# Autodesk Inventor assembly: HexTrayRed
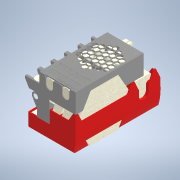
[picture p0: Inventor's stored thumbnail of the model, 180x180]
Saved by Autodesk Inventor 2021 (Build 250183000, 183)
## iProperties
Created: 2023-03-18
Part Number: HexTrayRed
Document SubType Name: Assembly
Designer: Bradley
Author: Bradley
## Documents named in this file (17)
- C:\Users\Bradley\Git\TI4\Hexes\HexTrayRed.iam
- C:\Users\Bradley\Git\TI4\Components\Hex_Hyperlanes_All.ipt
- C:\Users\Bradley\Git\TI4\Components\Hex_Mecatol.ipt
- C:\Users\Bradley\Git\TI4\Components\Hex_Reds_All.ipt
- C:\Users\Bradley\Git\TI4\Hexes\HexTrayRed.ipt
- C:\Users\Bradley\Git\TI4\Components\ActionCards_All.ipt
- C:\Users\Bradley\Git\TI4\Components\Exploration_SingleType.ipt
- C:\Users\Bradley\Git\TI4\Components\Objects_Public_SingleType.ipt
- C:\Users\Bradley\Git\TI4\Components\Objects_Secret_All.ipt
- C:\Users\Bradley\Git\TI4\Components\Relics_All.ipt
- C:\Users\Bradley\Git\TI4\Components\Planets_All.ipt
- C:\Users\Bradley\Git\TI4\Components\Agendas_All.ipt
- C:\Users\Bradley\Git\TI4\Hexes\HexTrayRed_Insert.ipt
- C:\Users\Bradley\Git\TI4\Hexes\CardboardTray.ipt
- C:\Users\Bradley\Git\TI4\Components\Cardboard_1_Single.ipt
- C:\Users\Bradley\Git\TI4\Components\Cardboard_3_Single.ipt
- C:\Users\Bradley\Git\TI4\Hexes\CardboardTray_Lid2.ipt
## Components (205 placed, 16 different names)
1. CardboardTray:1 — Mate:41, Flush:21, Flush:22, Insert:1, Insert:44, Insert:45, Insert:46, Insert:47, Insert:48, Insert:49, Mate:42, Mate:43, Mate:44, Mate:45, Mate:46, Mate:47, Mate:48, Mate:49, Mate:50, Mate:51, Mate:52, Mate:53, Mate:54, Mate:55, Mate:56, Mate:57, Mate:58, Mate:59, Mate:60, Mate:61, Mate:62
2. HexTrayRed:1 — Mate:2, Mate:3, Flush:3, Mate:4, Mate:11, Mate:12, Mate:13, Mate:16, Mate:17, Mate:18, Mate:19, Mate:20, Mate:21, Mate:22, Mate:23, Mate:24, Mate:25, Mate:26, Mate:27, Mate:28, Mate:29, Mate:30, Mate:31, Mate:32, Mate:33, Flush:20, Mate:34, Mate:41, Flush:21, Flush:22
3. HexTrayRed_Insert:1 — Mate:33, Flush:20, Mate:34, Mate:35, Mate:36, Mate:37, Mate:38, Mate:39, Mate:40
4. CardboardTray_Lid2:1 — Mate:60, Mate:61, Mate:62
5. Agendas_All:1 — Mate:36, Mate:37, Mate:39
6. ActionCards_All:1 — Mate:19, Mate:20, Mate:21
7. Hex_Hyperlanes_All:1 — Mate:1, Flush:1, Flush:2, Flush:4, Flush:5, Mate:4
8. Hex_Mecatol:1 — Mate:1, Flush:1, Flush:2
9. Hex_Reds_All:1 — Mate:2, Mate:3, Flush:3, Flush:4, Flush:5
10. Objects_Public_SingleType:1 — Mate:16, Mate:17, Mate:18
11. Objects_Public_SingleType:2
12. Objects_Secret_All:1
13. Planets_All:1 — Mate:35, Mate:38, Mate:40
14. Relics_All:1 — Mate:31, Mate:32, Flush:19
15. Cardboard_1_Single:1 — Insert:50, Mate:42
16. Cardboard_1_Single:10
17. Cardboard_1_Single:100
18. Cardboard_1_Single:101
19. Cardboard_1_Single:102
20. Cardboard_1_Single:103
21. Cardboard_1_Single:104 — Mate:54
22. Cardboard_1_Single:105
23. Cardboard_1_Single:106
24. Cardboard_1_Single:107
25. Cardboard_1_Single:108 — Insert:150
26. Cardboard_1_Single:109 — Insert:150
27. Cardboard_1_Single:11
28. Cardboard_1_Single:110
29. Cardboard_1_Single:111
30. Cardboard_1_Single:112
31. Cardboard_1_Single:113
32. Cardboard_1_Single:114 — Mate:58
33. Cardboard_1_Single:115
34. Cardboard_1_Single:116
35. Cardboard_1_Single:117
36. Cardboard_1_Single:118
37. Cardboard_1_Single:119 — Mate:59
38. Cardboard_1_Single:120
39. Cardboard_1_Single:121
40. Cardboard_1_Single:122
41. Cardboard_1_Single:123
42. Cardboard_1_Single:124 — Mate:56
43. Cardboard_1_Single:125
44. Cardboard_1_Single:126
45. Cardboard_1_Single:127
46. Cardboard_1_Single:128
47. Cardboard_1_Single:129
48. Cardboard_1_Single:13 — Mate:44
49. Cardboard_1_Single:130
50. Cardboard_1_Single:131
51. Cardboard_1_Single:132
52. Cardboard_1_Single:133
53. Cardboard_1_Single:134 — Mate:57
54. Cardboard_1_Single:135
55. Cardboard_1_Single:136
56. Cardboard_1_Single:137
57. Cardboard_1_Single:138
58. Cardboard_1_Single:139
59. Cardboard_1_Single:14
60. Cardboard_1_Single:140
61. Cardboard_1_Single:141
62. Cardboard_1_Single:142
63. Cardboard_1_Single:143
64. Cardboard_1_Single:15
65. Cardboard_1_Single:16
66. Cardboard_1_Single:17
67. Cardboard_1_Single:19 — Mate:47
68. Cardboard_1_Single:2 — Insert:50, Insert:51
69. Cardboard_1_Single:20
70. Cardboard_1_Single:21
71. Cardboard_1_Single:22
72. Cardboard_1_Single:23
73. Cardboard_1_Single:25 — Mate:46
74. Cardboard_1_Single:26
75. Cardboard_1_Single:27
76. Cardboard_1_Single:28
77. Cardboard_1_Single:29
78. Cardboard_1_Single:3 — Insert:51, Insert:52
79. Cardboard_1_Single:31 — Mate:45
80. Cardboard_1_Single:32
81. Cardboard_1_Single:33
82. Cardboard_1_Single:34
83. Cardboard_1_Single:35
84. Cardboard_1_Single:37 — Mate:48
85. Cardboard_1_Single:38
86. Cardboard_1_Single:39
87. Cardboard_1_Single:4 — Insert:52, Insert:53
88. Cardboard_1_Single:40
89. Cardboard_1_Single:41
90. Cardboard_1_Single:43 — Mate:49
91. Cardboard_1_Single:44
92. Cardboard_1_Single:45
93. Cardboard_1_Single:46
94. Cardboard_1_Single:47
95. Cardboard_1_Single:49 — Mate:50
96. Cardboard_1_Single:5 — Insert:53
97. Cardboard_1_Single:50
98. Cardboard_1_Single:51
99. Cardboard_1_Single:52
100. Cardboard_1_Single:53
101. Cardboard_1_Single:54 — Mate:51
102. Cardboard_1_Single:55
103. Cardboard_1_Single:56
104. Cardboard_1_Single:57
105. Cardboard_1_Single:58 — Insert:104
106. Cardboard_1_Single:59 — Insert:105, Insert:106
107. Cardboard_1_Single:60 — Insert:104
108. Cardboard_1_Single:61
109. Cardboard_1_Single:62
110. Cardboard_1_Single:63
111. Cardboard_1_Single:64 — Insert:105
112. Cardboard_1_Single:65 — Insert:106, Insert:107
113. Cardboard_1_Single:66 — Insert:107, Insert:108
114. Cardboard_1_Single:67 — Insert:108, Insert:109
115. Cardboard_1_Single:68 — Insert:109
116. Cardboard_1_Single:69 — Mate:53
117. Cardboard_1_Single:7 — Mate:43
118. Cardboard_1_Single:70
119. Cardboard_1_Single:71
120. Cardboard_1_Single:72
121. Cardboard_1_Single:73
122. Cardboard_1_Single:74
123. Cardboard_1_Single:75
124. Cardboard_1_Single:76
125. Cardboard_1_Single:77
126. Cardboard_1_Single:78
127. Cardboard_1_Single:79
128. Cardboard_1_Single:8
129. Cardboard_1_Single:80
130. Cardboard_1_Single:81
131. Cardboard_1_Single:82
132. Cardboard_1_Single:83
133. Cardboard_1_Single:84 — Mate:52
134. Cardboard_1_Single:85
135. Cardboard_1_Single:86
136. Cardboard_1_Single:87
137. Cardboard_1_Single:88
138. Cardboard_1_Single:89
139. Cardboard_1_Single:9
140. Cardboard_1_Single:90
141. Cardboard_1_Single:91
142. Cardboard_1_Single:92
143. Cardboard_1_Single:93
144. Cardboard_1_Single:94
145. Cardboard_1_Single:95
146. Cardboard_1_Single:96
147. Cardboard_1_Single:97
148. Cardboard_1_Single:98
149. Cardboard_1_Single:99 — Mate:55
150. Cardboard_3_Single:1 — Insert:1, Insert:2
151. Cardboard_3_Single:10
152. Cardboard_3_Single:11
153. Cardboard_3_Single:12
154. Cardboard_3_Single:13
155. Cardboard_3_Single:14
156. Cardboard_3_Single:15
157. Cardboard_3_Single:16
158. Cardboard_3_Single:17 — Insert:45
159. Cardboard_3_Single:18
160. Cardboard_3_Single:19
161. Cardboard_3_Single:2 — Insert:2, Insert:3
162. Cardboard_3_Single:20
163. Cardboard_3_Single:21
164. Cardboard_3_Single:22
165. Cardboard_3_Single:23
166. Cardboard_3_Single:24
167. Cardboard_3_Single:25 — Insert:46
168. Cardboard_3_Single:26
169. Cardboard_3_Single:27
170. Cardboard_3_Single:28
171. Cardboard_3_Single:29
172. Cardboard_3_Single:3 — Insert:3, Insert:4
173. Cardboard_3_Single:30
174. Cardboard_3_Single:31
175. Cardboard_3_Single:32
176. Cardboard_3_Single:33 — Insert:47
177. Cardboard_3_Single:34
178. Cardboard_3_Single:35
179. Cardboard_3_Single:36
180. Cardboard_3_Single:37
181. Cardboard_3_Single:38
182. Cardboard_3_Single:39
183. Cardboard_3_Single:4 — Insert:4, Insert:5
184. Cardboard_3_Single:40
185. Cardboard_3_Single:41 — Insert:55
186. Cardboard_3_Single:42 — Insert:55
187. Cardboard_3_Single:43
188. Cardboard_3_Single:44 — Insert:48
189. Cardboard_3_Single:46 — Insert:56
190. Cardboard_3_Single:47
191. Cardboard_3_Single:48 — Insert:49
192. Cardboard_3_Single:49 — Insert:56
193. Cardboard_3_Single:5 — Insert:5, Insert:6
194. Cardboard_3_Single:6 — Insert:6, Insert:7
195. Cardboard_3_Single:7 — Insert:7, Insert:8
196. Cardboard_3_Single:8 — Insert:8
197. Cardboard_3_Single:9 — Insert:44
198. Exploration_SingleType:1 — Mate:11, Mate:12, Mate:13
199. Exploration_SingleType:2
200. Exploration_SingleType:3
201. Exploration_SingleType:4
202. Exploration_SingleType:5 — Mate:22, Mate:23, Mate:24, Flush:16
203. Exploration_SingleType:6 — Mate:25, Mate:26, Flush:16, Flush:17
204. Exploration_SingleType:7 — Mate:27, Mate:28, Flush:17, Flush:18
205. Exploration_SingleType:8 — Mate:29, Mate:30, Flush:18, Flush:19
## Relationships (246: Insert 165, Mate 59, Flush 22)
- Mate:1: Hex_Hyperlanes_All:1 ↔ Hex_Mecatol:1
- Flush:1: Hex_Hyperlanes_All:1 ↔ Hex_Mecatol:1
- Flush:2: Hex_Hyperlanes_All:1 ↔ Hex_Mecatol:1
- Mate:2 (0.3 mm): HexTrayRed:1 ↔ Hex_Reds_All:1
- Mate:3: HexTrayRed:1 ↔ Hex_Reds_All:1
- Flush:3: HexTrayRed:1 ↔ Hex_Reds_All:1
- Flush:4: Hex_Hyperlanes_All:1 ↔ Hex_Reds_All:1
- Flush:5: Hex_Hyperlanes_All:1 ↔ Hex_Reds_All:1
- Mate:4 (0.4 mm): HexTrayRed:1 ↔ Hex_Hyperlanes_All:1
- [Mate]: Exploration_SingleType:1 ↔ Exploration_SingleType:2
- [Mate]: Exploration_SingleType:2 ↔ Exploration_SingleType:3
- [Mate]: Exploration_SingleType:3 ↔ Exploration_SingleType:4
- [Flush]: Exploration_SingleType:3 ↔ Exploration_SingleType:4
- [Flush]: Exploration_SingleType:2 ↔ Exploration_SingleType:3
- [Flush]: Exploration_SingleType:1 ↔ Exploration_SingleType:2
- [Flush]: Exploration_SingleType:3 ↔ Exploration_SingleType:4
- [Flush]: Exploration_SingleType:2 ↔ Exploration_SingleType:3
- [Flush]: Exploration_SingleType:1 ↔ Exploration_SingleType:2
- Mate:11: HexTrayRed:1 ↔ Exploration_SingleType:1
- Mate:12 (0.5 mm): HexTrayRed:1 ↔ Exploration_SingleType:1
- Mate:13 (0.5 mm): HexTrayRed:1 ↔ Exploration_SingleType:1
- [Mate]: Objects_Public_SingleType:1 ↔ Objects_Public_SingleType:2
- [Mate]: Objects_Public_SingleType:2 ↔ Objects_Secret_All:1
- [Flush]: Objects_Public_SingleType:2 ↔ Objects_Secret_All:1
- [Flush]: Objects_Public_SingleType:1 ↔ Objects_Public_SingleType:2
- [Flush]: Objects_Public_SingleType:1 ↔ Objects_Public_SingleType:2
- [Flush]: Objects_Public_SingleType:2 ↔ Objects_Secret_All:1
- Mate:16: HexTrayRed:1 ↔ Objects_Public_SingleType:1
- Mate:17 (0.5 mm): HexTrayRed:1 ↔ Objects_Public_SingleType:1
- Mate:18 (0.5 mm): HexTrayRed:1 ↔ Objects_Public_SingleType:1
- Mate:19: HexTrayRed:1 ↔ ActionCards_All:1
- Mate:20 (0.5 mm): HexTrayRed:1 ↔ ActionCards_All:1
- Mate:21 (0.5 mm): HexTrayRed:1 ↔ ActionCards_All:1
- Mate:22: HexTrayRed:1 ↔ Exploration_SingleType:5
- Mate:23: HexTrayRed:1 ↔ Exploration_SingleType:5
- Mate:24 (0.5 mm): HexTrayRed:1 ↔ Exploration_SingleType:5
- Mate:25: HexTrayRed:1 ↔ Exploration_SingleType:6
- Mate:26: HexTrayRed:1 ↔ Exploration_SingleType:6
- Mate:27: HexTrayRed:1 ↔ Exploration_SingleType:7
- Mate:28: HexTrayRed:1 ↔ Exploration_SingleType:7
- Mate:29: HexTrayRed:1 ↔ Exploration_SingleType:8
- Mate:30: HexTrayRed:1 ↔ Exploration_SingleType:8
- Flush:16: Exploration_SingleType:5 ↔ Exploration_SingleType:6
- Flush:17: Exploration_SingleType:6 ↔ Exploration_SingleType:7
- Flush:18: Exploration_SingleType:7 ↔ Exploration_SingleType:8
- Mate:31: HexTrayRed:1 ↔ Relics_All:1
- Mate:32: HexTrayRed:1 ↔ Relics_All:1
- Flush:19: Relics_All:1 ↔ Exploration_SingleType:8
- Mate:33: HexTrayRed:1 ↔ HexTrayRed_Insert:1
- Flush:20: HexTrayRed:1 ↔ HexTrayRed_Insert:1
- Mate:34: HexTrayRed:1 ↔ HexTrayRed_Insert:1
- Mate:35: HexTrayRed_Insert:1 ↔ Planets_All:1
- Mate:36: HexTrayRed_Insert:1 ↔ Agendas_All:1
- Mate:37: HexTrayRed_Insert:1 ↔ Agendas_All:1
- Mate:38: HexTrayRed_Insert:1 ↔ Planets_All:1
- Mate:39 (0.5 mm): HexTrayRed_Insert:1 ↔ Agendas_All:1
- Mate:40 (0.5 mm): HexTrayRed_Insert:1 ↔ Planets_All:1
- Mate:41: CardboardTray:1 ↔ HexTrayRed:1
- Flush:21: CardboardTray:1 ↔ HexTrayRed:1
- Flush:22: CardboardTray:1 ↔ HexTrayRed:1
- Insert:1: CardboardTray:1 ↔ Cardboard_3_Single:1
- Insert:2: Cardboard_3_Single:1 ↔ Cardboard_3_Single:2
- Insert:3: Cardboard_3_Single:2 ↔ Cardboard_3_Single:3
- Insert:4: Cardboard_3_Single:3 ↔ Cardboard_3_Single:4
- Insert:5: Cardboard_3_Single:4 ↔ Cardboard_3_Single:5
- Insert:6: Cardboard_3_Single:5 ↔ Cardboard_3_Single:6
- Insert:7: Cardboard_3_Single:6 ↔ Cardboard_3_Single:7
- Insert:8: Cardboard_3_Single:7 ↔ Cardboard_3_Single:8
- [Insert]: Cardboard_3_Single:10 ↔ Cardboard_3_Single:9
- [Insert]: Cardboard_3_Single:10 ↔ Cardboard_3_Single:11
- [Insert]: Cardboard_3_Single:11 ↔ Cardboard_3_Single:12
- [Insert]: Cardboard_3_Single:12 ↔ Cardboard_3_Single:13
- [Insert]: Cardboard_3_Single:13 ↔ Cardboard_3_Single:14
- [Insert]: Cardboard_3_Single:14 ↔ Cardboard_3_Single:15
- [Insert]: Cardboard_3_Single:15 ↔ Cardboard_3_Single:16
- [Insert]: Cardboard_3_Single:17 ↔ Cardboard_3_Single:18
- [Insert]: Cardboard_3_Single:18 ↔ Cardboard_3_Single:19
- [Insert]: Cardboard_3_Single:19 ↔ Cardboard_3_Single:20
- [Insert]: Cardboard_3_Single:20 ↔ Cardboard_3_Single:21
- [Insert]: Cardboard_3_Single:21 ↔ Cardboard_3_Single:22
- [Insert]: Cardboard_3_Single:22 ↔ Cardboard_3_Single:23
- [Insert]: Cardboard_3_Single:23 ↔ Cardboard_3_Single:24
- [Insert]: Cardboard_3_Single:25 ↔ Cardboard_3_Single:26
- [Insert]: Cardboard_3_Single:26 ↔ Cardboard_3_Single:27
- [Insert]: Cardboard_3_Single:27 ↔ Cardboard_3_Single:28
- [Insert]: Cardboard_3_Single:28 ↔ Cardboard_3_Single:29
- [Insert]: Cardboard_3_Single:29 ↔ Cardboard_3_Single:30
- [Insert]: Cardboard_3_Single:30 ↔ Cardboard_3_Single:31
- [Insert]: Cardboard_3_Single:31 ↔ Cardboard_3_Single:32
- [Insert]: Cardboard_3_Single:33 ↔ Cardboard_3_Single:34
- [Insert]: Cardboard_3_Single:34 ↔ Cardboard_3_Single:35
- [Insert]: Cardboard_3_Single:35 ↔ Cardboard_3_Single:36
- [Insert]: Cardboard_3_Single:36 ↔ Cardboard_3_Single:37
- [Insert]: Cardboard_3_Single:37 ↔ Cardboard_3_Single:38
- [Insert]: Cardboard_3_Single:38 ↔ Cardboard_3_Single:39
- [Insert]: Cardboard_3_Single:39 ↔ Cardboard_3_Single:40
- [Insert]: Cardboard_3_Single:42 ↔ Cardboard_3_Single:43
- [Insert]: Cardboard_3_Single:43 ↔ Cardboard_3_Single:44
- [Insert]: Cardboard_3_Single:46 ↔ Cardboard_3_Single:47
- [Insert]: Cardboard_3_Single:47 ↔ Cardboard_3_Single:48
- Insert:44: CardboardTray:1 ↔ Cardboard_3_Single:9
- Insert:45: CardboardTray:1 ↔ Cardboard_3_Single:17
- Insert:46: CardboardTray:1 ↔ Cardboard_3_Single:25
- Insert:47: CardboardTray:1 ↔ Cardboard_3_Single:33
- Insert:48 (0.5 mm): CardboardTray:1 ↔ Cardboard_3_Single:44
- Insert:49 (0.5 mm): CardboardTray:1 ↔ Cardboard_3_Single:48
- Insert:50: Cardboard_1_Single:1 ↔ Cardboard_1_Single:2
- Insert:51: Cardboard_1_Single:2 ↔ Cardboard_1_Single:3
- Insert:52: Cardboard_1_Single:3 ↔ Cardboard_1_Single:4
- Insert:53: Cardboard_1_Single:4 ↔ Cardboard_1_Single:5
- Insert:55: Cardboard_3_Single:41 ↔ Cardboard_3_Single:42
- Insert:56: Cardboard_3_Single:46 ↔ Cardboard_3_Single:49
- Mate:42: CardboardTray:1 ↔ Cardboard_1_Single:1
- [Insert]: Cardboard_1_Single:7 ↔ Cardboard_1_Single:8
- [Insert]: Cardboard_1_Single:8 ↔ Cardboard_1_Single:9
- [Insert]: Cardboard_1_Single:10 ↔ Cardboard_1_Single:9
- [Insert]: Cardboard_1_Single:10 ↔ Cardboard_1_Single:11
- [Insert]: Cardboard_1_Single:13 ↔ Cardboard_1_Single:14
- [Insert]: Cardboard_1_Single:14 ↔ Cardboard_1_Single:15
- [Insert]: Cardboard_1_Single:15 ↔ Cardboard_1_Single:16
- [Insert]: Cardboard_1_Single:16 ↔ Cardboard_1_Single:17
- [Insert]: Cardboard_1_Single:19 ↔ Cardboard_1_Single:20
- [Insert]: Cardboard_1_Single:20 ↔ Cardboard_1_Single:21
- [Insert]: Cardboard_1_Single:21 ↔ Cardboard_1_Single:22
- [Insert]: Cardboard_1_Single:22 ↔ Cardboard_1_Single:23
- [Insert]: Cardboard_1_Single:25 ↔ Cardboard_1_Single:26
- [Insert]: Cardboard_1_Single:26 ↔ Cardboard_1_Single:27
- [Insert]: Cardboard_1_Single:27 ↔ Cardboard_1_Single:28
- [Insert]: Cardboard_1_Single:28 ↔ Cardboard_1_Single:29
- [Insert]: Cardboard_1_Single:31 ↔ Cardboard_1_Single:32
- [Insert]: Cardboard_1_Single:32 ↔ Cardboard_1_Single:33
- [Insert]: Cardboard_1_Single:33 ↔ Cardboard_1_Single:34
- [Insert]: Cardboard_1_Single:34 ↔ Cardboard_1_Single:35
- [Insert]: Cardboard_1_Single:37 ↔ Cardboard_1_Single:38
- [Insert]: Cardboard_1_Single:38 ↔ Cardboard_1_Single:39
- [Insert]: Cardboard_1_Single:39 ↔ Cardboard_1_Single:40
- [Insert]: Cardboard_1_Single:40 ↔ Cardboard_1_Single:41
- [Insert]: Cardboard_1_Single:43 ↔ Cardboard_1_Single:44
- [Insert]: Cardboard_1_Single:44 ↔ Cardboard_1_Single:45
- [Insert]: Cardboard_1_Single:45 ↔ Cardboard_1_Single:46
- [Insert]: Cardboard_1_Single:46 ↔ Cardboard_1_Single:47
- [Insert]: Cardboard_1_Single:49 ↔ Cardboard_1_Single:50
- [Insert]: Cardboard_1_Single:50 ↔ Cardboard_1_Single:51
- [Insert]: Cardboard_1_Single:51 ↔ Cardboard_1_Single:52
- [Insert]: Cardboard_1_Single:52 ↔ Cardboard_1_Single:53
- Mate:43: CardboardTray:1 ↔ Cardboard_1_Single:7
- Mate:44: CardboardTray:1 ↔ Cardboard_1_Single:13
- Mate:45: CardboardTray:1 ↔ Cardboard_1_Single:31
- Mate:46: CardboardTray:1 ↔ Cardboard_1_Single:25
- Mate:47: CardboardTray:1 ↔ Cardboard_1_Single:19
- Mate:48: CardboardTray:1 ↔ Cardboard_1_Single:37
- Mate:49: CardboardTray:1 ↔ Cardboard_1_Single:43
- Mate:50: CardboardTray:1 ↔ Cardboard_1_Single:49
- [Insert]: Cardboard_1_Single:54 ↔ Cardboard_1_Single:55
- [Insert]: Cardboard_1_Single:55 ↔ Cardboard_1_Single:56
- [Insert]: Cardboard_1_Single:56 ↔ Cardboard_1_Single:57
- [Insert]: Cardboard_1_Single:57 ↔ Cardboard_1_Single:58
- [Insert]: Cardboard_1_Single:60 ↔ Cardboard_1_Single:61
- [Insert]: Cardboard_1_Single:61 ↔ Cardboard_1_Single:62
- [Insert]: Cardboard_1_Single:62 ↔ Cardboard_1_Single:63
- [Insert]: Cardboard_1_Single:63 ↔ Cardboard_1_Single:64
- Insert:104: Cardboard_1_Single:58 ↔ Cardboard_1_Single:60
- Insert:105: Cardboard_1_Single:59 ↔ Cardboard_1_Single:64
- Insert:106: Cardboard_1_Single:59 ↔ Cardboard_1_Single:65
- Insert:107: Cardboard_1_Single:65 ↔ Cardboard_1_Single:66
- Insert:108: Cardboard_1_Single:66 ↔ Cardboard_1_Single:67
- Insert:109: Cardboard_1_Single:67 ↔ Cardboard_1_Single:68
- Mate:51: CardboardTray:1 ↔ Cardboard_1_Single:54
- [Insert]: Cardboard_1_Single:69 ↔ Cardboard_1_Single:70
- [Insert]: Cardboard_1_Single:70 ↔ Cardboard_1_Single:71
- [Insert]: Cardboard_1_Single:71 ↔ Cardboard_1_Single:72
- [Insert]: Cardboard_1_Single:72 ↔ Cardboard_1_Single:73
- [Insert]: Cardboard_1_Single:75 ↔ Cardboard_1_Single:76
- [Insert]: Cardboard_1_Single:76 ↔ Cardboard_1_Single:77
- [Insert]: Cardboard_1_Single:77 ↔ Cardboard_1_Single:78
- [Insert]: Cardboard_1_Single:78 ↔ Cardboard_1_Single:79
- [Insert]: Cardboard_1_Single:73 ↔ Cardboard_1_Single:75
- [Insert]: Cardboard_1_Single:74 ↔ Cardboard_1_Single:79
- [Insert]: Cardboard_1_Single:74 ↔ Cardboard_1_Single:80
- [Insert]: Cardboard_1_Single:80 ↔ Cardboard_1_Single:81
- [Insert]: Cardboard_1_Single:81 ↔ Cardboard_1_Single:82
- [Insert]: Cardboard_1_Single:82 ↔ Cardboard_1_Single:83
- [Insert]: Cardboard_1_Single:84 ↔ Cardboard_1_Single:85
- [Insert]: Cardboard_1_Single:85 ↔ Cardboard_1_Single:86
- [Insert]: Cardboard_1_Single:86 ↔ Cardboard_1_Single:87
- [Insert]: Cardboard_1_Single:87 ↔ Cardboard_1_Single:88
- [Insert]: Cardboard_1_Single:90 ↔ Cardboard_1_Single:91
- [Insert]: Cardboard_1_Single:91 ↔ Cardboard_1_Single:92
- [Insert]: Cardboard_1_Single:92 ↔ Cardboard_1_Single:93
- [Insert]: Cardboard_1_Single:93 ↔ Cardboard_1_Single:94
- [Insert]: Cardboard_1_Single:88 ↔ Cardboard_1_Single:90
- [Insert]: Cardboard_1_Single:89 ↔ Cardboard_1_Single:94
- [Insert]: Cardboard_1_Single:89 ↔ Cardboard_1_Single:95
- [Insert]: Cardboard_1_Single:95 ↔ Cardboard_1_Single:96
- [Insert]: Cardboard_1_Single:96 ↔ Cardboard_1_Single:97
- [Insert]: Cardboard_1_Single:97 ↔ Cardboard_1_Single:98
- Mate:52: CardboardTray:1 ↔ Cardboard_1_Single:84
- Mate:53: CardboardTray:1 ↔ Cardboard_1_Single:69
- [Insert]: Cardboard_1_Single:100 ↔ Cardboard_1_Single:99
- [Insert]: Cardboard_1_Single:100 ↔ Cardboard_1_Single:101
- [Insert]: Cardboard_1_Single:101 ↔ Cardboard_1_Single:102
- [Insert]: Cardboard_1_Single:102 ↔ Cardboard_1_Single:103
- [Insert]: Cardboard_1_Single:104 ↔ Cardboard_1_Single:105
- [Insert]: Cardboard_1_Single:105 ↔ Cardboard_1_Single:106
- [Insert]: Cardboard_1_Single:106 ↔ Cardboard_1_Single:107
- [Insert]: Cardboard_1_Single:107 ↔ Cardboard_1_Single:108
- [Insert]: Cardboard_1_Single:109 ↔ Cardboard_1_Single:110
- [Insert]: Cardboard_1_Single:110 ↔ Cardboard_1_Single:111
- [Insert]: Cardboard_1_Single:111 ↔ Cardboard_1_Single:112
- [Insert]: Cardboard_1_Single:112 ↔ Cardboard_1_Single:113
- Insert:150: Cardboard_1_Single:108 ↔ Cardboard_1_Single:109
- Mate:54: CardboardTray:1 ↔ Cardboard_1_Single:104
- Mate:55: CardboardTray:1 ↔ Cardboard_1_Single:99
- [Insert]: Cardboard_1_Single:114 ↔ Cardboard_1_Single:115
- [Insert]: Cardboard_1_Single:115 ↔ Cardboard_1_Single:116
- [Insert]: Cardboard_1_Single:116 ↔ Cardboard_1_Single:117
- [Insert]: Cardboard_1_Single:117 ↔ Cardboard_1_Single:118
- [Insert]: Cardboard_1_Single:119 ↔ Cardboard_1_Single:120
- [Insert]: Cardboard_1_Single:120 ↔ Cardboard_1_Single:121
- [Insert]: Cardboard_1_Single:121 ↔ Cardboard_1_Single:122
- [Insert]: Cardboard_1_Single:122 ↔ Cardboard_1_Single:123
- [Insert]: Cardboard_1_Single:124 ↔ Cardboard_1_Single:125
- [Insert]: Cardboard_1_Single:125 ↔ Cardboard_1_Single:126
- [Insert]: Cardboard_1_Single:126 ↔ Cardboard_1_Single:127
- [Insert]: Cardboard_1_Single:127 ↔ Cardboard_1_Single:128
- [Insert]: Cardboard_1_Single:129 ↔ Cardboard_1_Single:130
- [Insert]: Cardboard_1_Single:130 ↔ Cardboard_1_Single:131
- [Insert]: Cardboard_1_Single:131 ↔ Cardboard_1_Single:132
- [Insert]: Cardboard_1_Single:132 ↔ Cardboard_1_Single:133
- [Insert]: Cardboard_1_Single:128 ↔ Cardboard_1_Single:129
- [Insert]: Cardboard_1_Single:134 ↔ Cardboard_1_Single:135
- [Insert]: Cardboard_1_Single:135 ↔ Cardboard_1_Single:136
- [Insert]: Cardboard_1_Single:136 ↔ Cardboard_1_Single:137
- [Insert]: Cardboard_1_Single:137 ↔ Cardboard_1_Single:138
- [Insert]: Cardboard_1_Single:139 ↔ Cardboard_1_Single:140
- [Insert]: Cardboard_1_Single:140 ↔ Cardboard_1_Single:141
- [Insert]: Cardboard_1_Single:141 ↔ Cardboard_1_Single:142
- [Insert]: Cardboard_1_Single:142 ↔ Cardboard_1_Single:143
- [Insert]: Cardboard_1_Single:138 ↔ Cardboard_1_Single:139
- Mate:56: CardboardTray:1 ↔ Cardboard_1_Single:124
- Mate:57: CardboardTray:1 ↔ Cardboard_1_Single:134
- Mate:58: CardboardTray:1 ↔ Cardboard_1_Single:114
- Mate:59: CardboardTray:1 ↔ Cardboard_1_Single:119
- Mate:60: CardboardTray:1 ↔ CardboardTray_Lid2:1
- Mate:61: CardboardTray:1 ↔ CardboardTray_Lid2:1
- Mate:62 (0.08 mm): CardboardTray:1 ↔ CardboardTray_Lid2:1
## Named parameters: d91_d84 = 0 mm, d92_d85 = 0 mm, d93_d86 = 0 mm, d94_d87 = 0 mm, d95_d88 = 0 mm, d96_d89 = 0 mm, d97_d90 = 0 mm, d98_d84 = 0 mm, d99_d85 = 0 mm, d100_d86 = 0 mm, d101_d87 = 0 mm, d102_d88 = 0 mm, d103_d89 = 0 mm, d104_d90 = 0 mm, d105_d84 = 0 mm, d106_d85 = 0 mm, d107_d86 = 0 mm, d108_d87 = 0 mm, d109_d88 = 0 mm, d110_d89 = 0 mm, d111_d90 = 0 mm, d112_d84 = 0 mm, d113_d85 = 0 mm, d114_d86 = 0 mm, d115_d87 = 0 mm, d116_d88 = 0 mm, d117_d89 = 0 mm, d118_d90 = 0 mm, d120_d85 = 0 mm, d121_d86 = 0 mm, d124_d89 = 0 mm, d125_d90 = 0 mm, d141_d132 = 0 mm, d142_d133 = 0 mm, d143_d134 = 0 mm, d144_d135 = 0 mm, d146_d132 = 0 mm, d147_d133 = 0 mm, d148_d134 = 0 mm, d149_d135 = 0 mm, d151_d132 = 0 mm, d152_d133 = 0 mm, d153_d134 = 0 mm, d154_d135 = 0 mm, d156_d132 = 0 mm, d157_d133 = 0 mm, d158_d134 = 0 mm, d159_d135 = 0 mm, d161_d132 = 0 mm, d162_d133 = 0 mm, d163_d134 = 0 mm, d164_d135 = 0 mm, d166_d132 = 0 mm, d167_d133 = 0 mm, d168_d134 = 0 mm, d169_d135 = 0 mm, d171_d132 = 0 mm, d172_d133 = 0 mm, d173_d134 = 0 mm, d174_d135 = 0 mm, d176_d132 = 0 mm, d177_d133 = 0 mm, d178_d134 = 0 mm, d179_d135 = 0 mm, d189_d132 = 0 mm, d190_d133 = 0 mm, d191_d134 = 0 mm, d192_d135 = 0 mm, d193_d132 = 0 mm, d194_d133 = 0 mm, d195_d134 = 0 mm, d196_d135 = 0 mm, d204_d193_d132 = 0 mm, d205_d194_d133 = 0 mm, d206_d195_d134 = 0 mm, d207_d196_d135 = 0 mm, d208_d197 = 0 mm, d209_d198 = 0 mm, d210_d199 = 0 mm, d211_d200 = 0 mm, d212_d201 = 0 mm, d213_d202 = 0 mm, d214_d189_d132 = 0 mm, d215_d190_d133 = 0 mm, d216_d191_d134 = 0 mm, d217_d192_d135 = 0 mm, d218_d193_d132 = 0 mm, d219_d194_d133 = 0 mm, d220_d195_d134 = 0 mm, d221_d196_d135 = 0 mm, d222_d197 = 0 mm, d223_d198 = 0 mm, d224_d199 = 0 mm, d225_d200 = 0 mm, d226_d201 = 0 mm, d227_d202 = 0 mm, d228_d189_d132 = 0 mm, d229_d190_d133 = 0 mm, d230_d191_d134 = 0 mm, d231_d192_d135 = 0 mm, d234_d146_d132 = 0 mm, d235_d147_d133 = 0 mm, d236_d148_d134 = 0 mm, d237_d149_d135 = 0 mm, d238_d146_d132 = 0 mm, d239_d147_d133 = 0 mm, d240_d148_d134 = 0 mm, d241_d149_d135 = 0 mm, d242_d146_d132 = 0 mm, d243_d147_d133 = 0 mm, d244_d148_d134 = 0 mm, d245_d149_d135 = 0 mm, d249_d234_d146_d132 = 0 mm, d250_d235_d147_d133 = 0 mm, d251_d236_d148_d134 = 0 mm, d252_d237_d149_d135 = 0 mm, d253_d234_d146_d132 = 0 mm, d254_d235_d147_d133 = 0 mm, d255_d236_d148_d134 = 0 mm, d256_d237_d149_d135 = 0 mm, d257_d238_d146_d132 = 0 mm, d258_d239_d147_d133 = 0 mm, d259_d240_d148_d134 = 0 mm, d260_d241_d149_d135 = 0 mm, d261_d242_d146_d132 = 0 mm, d262_d243_d147_d133 = 0 mm, d263_d244_d148_d134 = 0 mm, d264_d245_d149_d135 = 0 mm, d265_d246 = 0 mm, d266_d238_d146_d132 = 0 mm, d267_d239_d147_d133 = 0 mm, d268_d240_d148_d134 = 0 mm, d269_d241_d149_d135 = 0 mm, d270_d242_d146_d132 = 0 mm, d271_d243_d147_d133 = 0 mm, d272_d244_d148_d134 = 0 mm, d273_d245_d149_d135 = 0 mm, d274_d246 = 0 mm
